# Autodesk Inventor assembly: 45deg_mirror_assembly
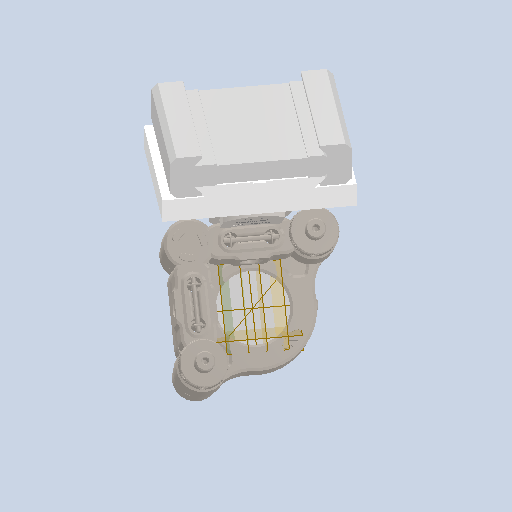
[picture p0: Inventor's stored thumbnail of the model, 512x512]
Saved by Autodesk Inventor 2026.1 (Build 301233000, 233)
## iProperties
Created: 2019-05-24
Part Number: 45deg_mirror_assembly
Document SubType Name: Assembly
Designer: Julian
Author: Julian
## Documents named in this file (5)
- C:\Users\user\Desktop\setup for publishing\45deg_mirror_assembly.iam
- C:\Users\user\Desktop\setup for publishing\rail_mount.iam
- C:\Users\user\Desktop\setup for publishing\POLARIS-MA45-45deg_mirror_mount.ipt
- C:\Users\user\Desktop\setup for publishing\SS100-F2H_suprema_1in_mirror_mount.ipt
- C:\Users\user\Desktop\setup for publishing\1in_5mm_mir.ipt
## Components (4 placed, 4 different names)
1. rail_mount:1 [sub-assembly] — Passend:1, Passend:2, Winkel:2
2. POLARIS-MA45-45deg_mirror_mount:1 — Passend:1, Passend:2, Passend:3, Passend:4
3. SS100-F2H_suprema_1in_mirror_mount:1 — Passend:3, Passend:4, Passend:5, Passend:6, Winkel:1
4. 1in_5mm_mir:1 — Passend:5, Passend:6, Winkel:1, Winkel:2
## Relationships (8: Mate 6, Angle 2)
- Passend:1 [Mate]: rail_mount:1 ↔ POLARIS-MA45-45deg_mirror_mount:1
- Passend:2 [Mate]: rail_mount:1 ↔ POLARIS-MA45-45deg_mirror_mount:1
- Passend:3 [Mate]: POLARIS-MA45-45deg_mirror_mount:1 ↔ SS100-F2H_suprema_1in_mirror_mount:1
- Passend:4 [Mate]: POLARIS-MA45-45deg_mirror_mount:1 ↔ SS100-F2H_suprema_1in_mirror_mount:1
- Passend:5 [Mate]: SS100-F2H_suprema_1in_mirror_mount:1 ↔ 1in_5mm_mir:1
- Passend:6 [Mate]: SS100-F2H_suprema_1in_mirror_mount:1 ↔ 1in_5mm_mir:1
- Winkel:1 [Angle] (0 deg): SS100-F2H_suprema_1in_mirror_mount:1 ↔ 1in_5mm_mir:1
- Winkel:2 [Angle] (180 deg): rail_mount:1 ↔ 1in_5mm_mir:1
